# Autodesk Inventor assembly: montagem_final_v2
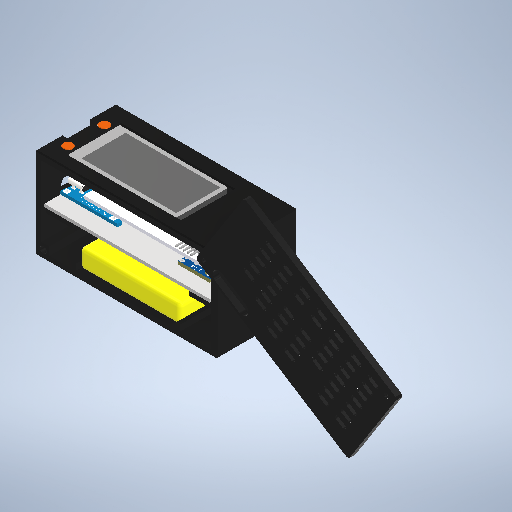
[picture p0: Inventor's stored thumbnail of the model, 512x512]
Saved by Autodesk Inventor 2025 (Build 290162000, 162)
## iProperties
Created: 2026-05-19
Part Number: montagem_final_v2
Document SubType Name: Assembly
Designer: pedro
Author: pedro
## Documents named in this file (7)
- C:\Users\pedro\OneDrive\Área de Trabalho\PEDRO\TCC - Eng. Controle e Automação\Prototipo peças\Prototipo Final\montagem_final_v2.iam
- C:\Users\pedro\OneDrive\Área de Trabalho\PEDRO\TCC - Eng. Controle e Automação\Prototipo peças\Prototipo Final\botão final.ipt
- C:\Users\pedro\OneDrive\Área de Trabalho\PEDRO\TCC - Eng. Controle e Automação\Prototipo peças\Prototipo Final\carcaça final.ipt
- C:\Users\pedro\OneDrive\Área de Trabalho\PEDRO\TCC - Eng. Controle e Automação\Prototipo peças\Prototipo Final\tampa final.ipt
- C:\Users\pedro\OneDrive\Área de Trabalho\PEDRO\TCC - Eng. Controle e Automação\Prototipo peças\Protótipo Inicial\bateria.ipt
- C:\Users\pedro\OneDrive\Área de Trabalho\PEDRO\TCC - Eng. Controle e Automação\Prototipo peças\Protótipo Esboço\montagem reg e carre.iam
- C:\Users\pedro\OneDrive\Área de Trabalho\PEDRO\TCC - Eng. Controle e Automação\Prototipo peças\Protótipo Esboço\montagem esp.iam
## Components (7 placed, 6 different names)
1. botão final:1 — Coincidente:1, Inserir:1
2. carcaça final:1 — Coincidente:1, Inserir:1, Coincidente:2, Inserir:2, Coincidente:3, Coincidente:4, Coincidente:5, Coincidente:7, Coincidente:8, Inserir:3
3. tampa final:1 — Inserir:3
4. botão final:2 — Coincidente:2, Inserir:2
5. bateria:1 — Coincidente:3, Coincidente:4, Coincidente:5
6. montagem reg e carre:1 [sub-assembly] — Coincidente:7, Coincidente:8
7. montagem esp:1 [sub-assembly]
## Relationships (10: Mate 7, Insert 3)
- Coincidente:1 [Mate]: botão final:1 ↔ carcaça final:1
- Inserir:1: botão final:1 ↔ carcaça final:1
- Coincidente:2 [Mate]: carcaça final:1 ↔ botão final:2
- Inserir:2: carcaça final:1 ↔ botão final:2
- Coincidente:3 [Mate]: carcaça final:1 ↔ bateria:1
- Coincidente:4 [Mate]: carcaça final:1 ↔ bateria:1
- Coincidente:5 [Mate]: carcaça final:1 ↔ bateria:1
- Coincidente:7 [Mate]: carcaça final:1 ↔ montagem reg e carre:1
- Coincidente:8 [Mate]: carcaça final:1 ↔ montagem reg e carre:1
- Inserir:3: carcaça final:1 ↔ tampa final:1
